# Autodesk Inventor assembly: 40cm
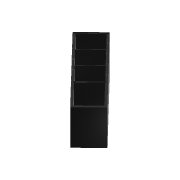
[picture p0: Inventor's stored thumbnail of the model, 180x180]
Saved by Autodesk Inventor 2020 (Build 240168000, 168)
## iProperties
Created: 2021-09-03
Part Number: 40cm
Document SubType Name: Assembly
Designer: Julian Uhl
Author: Julian Uhl
## Documents named in this file (6)
- C:\Schule\Eier-Inventor\40cm.iam
- C:\Schule\Eier-Inventor\3Eier_größer.ipt
- C:\Schule\Eier-Inventor\Raspberry_Dummy.ipt
- C:\Schule\Eier-Inventor\Ei_groß.ipt
- C:\Schule\Eier-Inventor\Ei.ipt
- C:\Schule\Eier-Inventor\Eihalter.ipt
## Components (8 placed, 5 different names)
1. 3Eier_größer:1 — Passend:12, Passend:13, Passend:14, Passend:15, Passend:16, Passend:17, Passend:18, Passend:19, Passend:20, Passend:21, Passend:22, Passend:23
2. Raspberry_Dummy:1 — Passend:12, Passend:13, Passend:14
3. Eihalter:1 — Passend:15, Passend:16, Passend:17
4. Eihalter:2 — Passend:18, Passend:19, Passend:20
5. Eihalter:3 — Passend:21, Passend:22, Passend:23
6. Ei:1
7. Ei_groß:2
8. Ei_groß:1
## Relationships (12: Mate 12)
- Passend:12 [Mate]: 3Eier_größer:1 ↔ Raspberry_Dummy:1
- Passend:13 [Mate] (20 mm): 3Eier_größer:1 ↔ Raspberry_Dummy:1
- Passend:14 [Mate] (20 mm): 3Eier_größer:1 ↔ Raspberry_Dummy:1
- Passend:15 [Mate] (100 mm): 3Eier_größer:1 ↔ Eihalter:1
- Passend:16 [Mate]: 3Eier_größer:1 ↔ Eihalter:1
- Passend:17 [Mate]: 3Eier_größer:1 ↔ Eihalter:1
- Passend:18 [Mate] (100 mm): 3Eier_größer:1 ↔ Eihalter:2
- Passend:19 [Mate]: 3Eier_größer:1 ↔ Eihalter:2
- Passend:20 [Mate]: 3Eier_größer:1 ↔ Eihalter:2
- Passend:21 [Mate] (100 mm): 3Eier_größer:1 ↔ Eihalter:3
- Passend:22 [Mate]: 3Eier_größer:1 ↔ Eihalter:3
- Passend:23 [Mate]: 3Eier_größer:1 ↔ Eihalter:3
